# Autodesk Inventor assembly: Leg
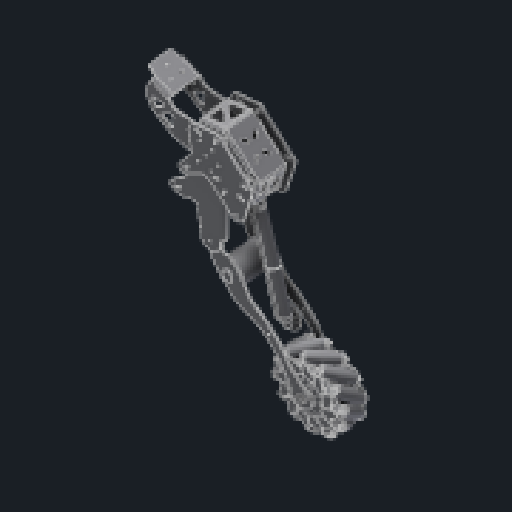
[picture p0: Inventor's stored thumbnail of the model, 512x512]
Saved by Autodesk Inventor 2025.2 (Build 292293000, 293)
## iProperties
Created: 2020-05-17
Part Number: Leg
Document SubType Name: Assembly
Designer: valer
Author: valer
## Documents named in this file (11)
- C:\Users\valer\Desktop\str1ker\cad\Leg.iam
- C:\Users\valer\Desktop\str1ker\cad\Knee.ipt
- C:\Users\valer\Desktop\str1ker\cad\LowerLeg.ipt
- C:\Users\valer\Desktop\str1ker\cad\UpperLeg.ipt
- C:\Users\valer\Desktop\str1ker\cad\Hip.ipt
- C:\Users\valer\Desktop\str1ker\cad\HipCoverTop.ipt
- C:\Users\valer\Desktop\str1ker\cad\external\FA-RMS-15-12-4-Piston.ipt
- C:\Users\valer\Desktop\str1ker\cad\external\FA-RMS-15-12-4.ipt
- C:\Users\valer\Desktop\str1ker\cad\external\2796N15_Omni-Directional Wheel.ipt
- C:\Users\valer\Desktop\str1ker\cad\WheelSproketHub.ipt
- C:\Users\valer\Desktop\str1ker\cad\external\MY6812-12VDC-120W.ipt
## Components (13 placed, 10 different names)
1. Knee:1 — Flush:1, Mate:1, Mate:3, Mate:4, Mate:14
2. LowerLeg:1 — Mate:3, Mate:14, Mate:38, Mate:46, Mate:53
3. UpperLeg:1 — Flush:1, Mate:1, Mate:4, Mate:6, Mate:7, Mate:17, Mate:18, Symmetry:1
4. Hip:1 — Mate:6, Mate:7, Mate:12, Mate:13, Flush:5, Mate:39
5. Knee:2 — Mate:50, Mate:51, Angle:1
6. UpperLeg:2 — Mate:12, Mate:13, Symmetry:1, Mate:36
7. HipCoverTop:1 — Mate:17, Mate:18, Mate:39
8. FA-RMS-15-12-4-Piston:1 — Flush:4, Mate:35, Mate:52
9. FA-RMS-15-12-4:1 — Mate:35, Mate:36
10. 2796N15_Omni-Directional Wheel:1 — Flush:4, Mate:38, Flush:5, Mate:46, Mate:55
11. LowerLeg:2 — Mate:50, Mate:51, Mate:52, Mate:54, Mate:55
12. MY6812-12VDC-120W:1 — Angle:1, Mate:53, Mate:54
13. WheelSproketHub:1
## Relationships (29: Mate 23, Flush 4, Symmetry 1, Angle 1)
- Flush:1 (-5.08 mm): Knee:1 ↔ UpperLeg:1
- Mate:1: Knee:1 ↔ UpperLeg:1
- Mate:3: Knee:1 ↔ LowerLeg:1
- Mate:4: Knee:1 ↔ UpperLeg:1
- Mate:6: UpperLeg:1 ↔ Hip:1
- Mate:7: UpperLeg:1 ↔ Hip:1
- [Flush] (5.08 mm): Knee:2 ↔ UpperLeg:2
- [Mate]: Knee:2 ↔ UpperLeg:2
- [Mate]: Knee:2 ↔ UpperLeg:2
- Mate:12: Hip:1 ↔ UpperLeg:2
- Mate:13: Hip:1 ↔ UpperLeg:2
- Mate:14: Knee:1 ↔ LowerLeg:1
- Mate:17: UpperLeg:1 ↔ HipCoverTop:1
- Mate:18: UpperLeg:1 ↔ HipCoverTop:1
- Symmetry:1: UpperLeg:1 ↔ UpperLeg:2
- Flush:4: FA-RMS-15-12-4-Piston:1 ↔ 2796N15_Omni-Directional Wheel:1
- Mate:35: FA-RMS-15-12-4-Piston:1 ↔ FA-RMS-15-12-4:1
- Mate:36: UpperLeg:2 ↔ FA-RMS-15-12-4:1
- Mate:38: LowerLeg:1 ↔ 2796N15_Omni-Directional Wheel:1
- Flush:5: Hip:1 ↔ 2796N15_Omni-Directional Wheel:1
- Mate:39: Hip:1 ↔ HipCoverTop:1
- Mate:46: LowerLeg:1 ↔ 2796N15_Omni-Directional Wheel:1
- Mate:50: Knee:2 ↔ LowerLeg:2
- Mate:51: Knee:2 ↔ LowerLeg:2
- Mate:52: FA-RMS-15-12-4-Piston:1 ↔ LowerLeg:2
- Angle:1 (180 deg): Knee:2 ↔ MY6812-12VDC-120W:1
- Mate:53: LowerLeg:1 ↔ MY6812-12VDC-120W:1
- Mate:54: LowerLeg:2 ↔ MY6812-12VDC-120W:1
- Mate:55: 2796N15_Omni-Directional Wheel:1 ↔ LowerLeg:2
## Named parameters: d11_d0 = 5.08 mm, d12_d1 = 0 mm, d15_d5 = 0 mm
